# Autodesk Inventor assembly: Bot Assembly V2
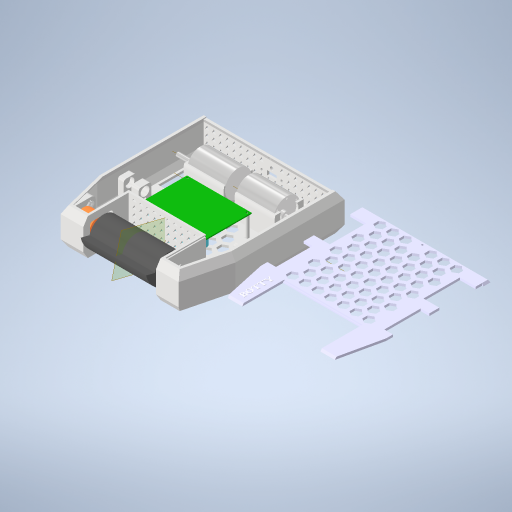
[picture p0: Inventor's stored thumbnail of the model, 512x512]
Saved by Autodesk Inventor 2024 (Build 280153000, 153)
## iProperties
Created: 2023-10-31
Part Number: Bot Assembly V2
Document SubType Name: Assembly
Designer: CJ110
Author: CJ110
## Documents named in this file (9)
- D:\GitHub\Vault-1\CAD\WCRL\Bot Assembly V2.iam
- D:\GitHub\Vault-1\CAD\WCRL\Bot v2 bottom.ipt
- D:\GitHub\Vault-1\CAD\WCRL\Brushless 2622 2600KV.ipt
- D:\GitHub\Vault-1\CAD\WCRL\Brushless Motor Mount.ipt
- D:\GitHub\Vault-1\CAD\WCRL\DC 12V 200RPM.ipt
- D:\GitHub\Vault-1\CAD\WCRL\Drum.ipt
- D:\GitHub\Vault-1\CAD\WCRL\LiPo.ipt
- D:\GitHub\Vault-1\CAD\WCRL\Bot v2 Top.ipt
- D:\GitHub\Vault-1\CAD\WCRL\PCB.ipt
## Components (9 placed, 8 different names)
1. Bot v2 bottom:1 — Mate:1, Mate:3, Mate:4, Mate:5, Mate:20, Mate:23, Mate:24, Mate:29, Mate:30, Mate:32, Mate:33, Mate:34, Mate:35, Mate:36, Mate:37, Mate:38
2. Brushless 2622 2600KV:1 — Mate:6, Mate:7, Mate:20
3. Brushless Motor Mount:1 — Mate:6, Mate:7, Mate:23, Mate:24
4. DC 12V 200RPM:1 — Mate:4, Mate:5
5. DC 12V 200RPM:2 — Mate:1, Mate:3
6. Drum:1 — Mate:37, Mate:38
7. LiPo:1 — Mate:33, Mate:34
8. PCB:1 — Mate:29, Mate:30, Mate:32
9. Bot v2 Top:2 — Mate:35, Mate:36
## Relationships (18: Mate 18)
- Mate:1: Bot v2 bottom:1 ↔ DC 12V 200RPM:2
- Mate:3: Bot v2 bottom:1 ↔ DC 12V 200RPM:2
- Mate:4: Bot v2 bottom:1 ↔ DC 12V 200RPM:1
- Mate:5: Bot v2 bottom:1 ↔ DC 12V 200RPM:1
- Mate:6: Brushless 2622 2600KV:1 ↔ Brushless Motor Mount:1
- Mate:7: Brushless 2622 2600KV:1 ↔ Brushless Motor Mount:1
- Mate:20: Bot v2 bottom:1 ↔ Brushless 2622 2600KV:1
- Mate:23: Bot v2 bottom:1 ↔ Brushless Motor Mount:1
- Mate:24: Bot v2 bottom:1 ↔ Brushless Motor Mount:1
- Mate:29: Bot v2 bottom:1 ↔ PCB:1
- Mate:30: Bot v2 bottom:1 ↔ PCB:1
- Mate:32: Bot v2 bottom:1 ↔ PCB:1
- Mate:33: Bot v2 bottom:1 ↔ LiPo:1
- Mate:34: Bot v2 bottom:1 ↔ LiPo:1
- Mate:35: Bot v2 bottom:1 ↔ Bot v2 Top:2
- Mate:36: Bot v2 bottom:1 ↔ Bot v2 Top:2
- Mate:37: Bot v2 bottom:1 ↔ Drum:1
- Mate:38: Bot v2 bottom:1 ↔ Drum:1
